# Autodesk Inventor assembly: byk
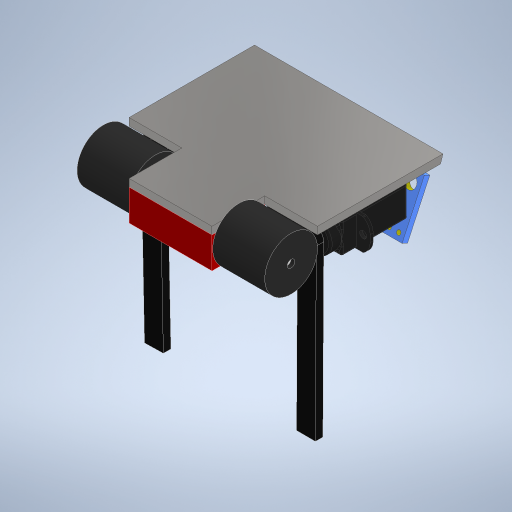
[picture p0: Inventor's stored thumbnail of the model, 512x512]
Saved by Autodesk Inventor 2023 (Build 270158000, 158)
## iProperties
Created: 2023-07-30
Part Number: byk
Document SubType Name: Assembly
Designer: Kamil
Author: Kamil
## Documents named in this file (10)
- C:\Users\Kamil\Documents\Inventor\MikroNalesnik\byk.iam
- C:\Users\Kamil\Documents\Inventor\MikroNalesnik\silnik_2.ipt
- C:\Users\Kamil\Documents\Inventor\MikroNalesnik\spod.ipt
- C:\Users\Kamil\Documents\Inventor\MikroNalesnik\TOF_VL53L0X (1).ipt
- C:\Users\Kamil\Documents\Inventor\MikroNalesnik\servo_mini_1370hd_cos.ipt
- C:\Users\Kamil\Documents\Inventor\MikroNalesnik\kolko.ipt
- C:\Users\Kamil\Documents\Inventor\MikroNalesnik\nozzz.ipt
- C:\Users\Kamil\Documents\Inventor\MikroNalesnik\wach.ipt
- C:\Users\Kamil\Documents\Inventor\MikroNalesnik\uchwyt silnikow.ipt
- C:\Users\Kamil\Documents\Inventor\MikroNalesnik\pcbb.ipt
## Components (15 placed, 9 different names)
1. silnik_2:2 — Zestawiające:21, Zestawiające:23, Zestawiające:25, Zestawiające:26, Zestawiające:27
2. spod:1 — Zestawiające:10, Zestawiające:11, Równoległe:6, Równoległe:7, Równoległe:8, Zestawiające:22, Zestawiające:24, Równoległe:9, Równoległe:12, Kątowe:1, Równoległe:18
3. TOF_VL53L0X (1):1 — Równoległe:3, Zestawiające:8, Równoległe:14, Równoległe:17
4. TOF_VL53L0X (1):2 — Równoległe:3, Równoległe:4, Zestawiające:8, Zestawiające:9, Kątowe:1, Równoległe:14, Równoległe:15, Równoległe:16, Równoległe:17
5. TOF_VL53L0X (1):3 — Równoległe:4, Zestawiające:9, Równoległe:15, Równoległe:16, Równoległe:18
6. servo_mini_1370hd_cos:1 — Zestawiające:10, Równoległe:5, Równoległe:8, Zestawiające:18, Zestawiające:19
7. servo_mini_1370hd_cos:2 — Zestawiające:11, Równoległe:5, Zestawiające:16, Zestawiające:17, Równoległe:7
8. kolko:1
9. nozzz:1 — Równoległe:6
10. wach:1 — Zestawiające:16, Zestawiające:17
11. wach:2 — Zestawiające:18, Zestawiające:19
12. silnik_2:3 — Zestawiające:21, Zestawiające:22, Zestawiające:23
13. kolko:2 — Zestawiające:26, Zestawiające:27
14. uchwyt silnikow:1 — Zestawiające:24, Zestawiające:25, Równoległe:9
15. pcbb:1 — Równoległe:12
## Relationships (29: Mate 15, Flush 13, Angle 1)
- Równoległe:3 [Flush]: TOF_VL53L0X (1):1 ↔ TOF_VL53L0X (1):2
- Równoległe:4 [Flush]: TOF_VL53L0X (1):2 ↔ TOF_VL53L0X (1):3
- Zestawiające:8 [Mate] (5 mm): TOF_VL53L0X (1):1 ↔ TOF_VL53L0X (1):2
- Zestawiające:9 [Mate] (5 mm): TOF_VL53L0X (1):2 ↔ TOF_VL53L0X (1):3
- Zestawiające:10 [Mate]: spod:1 ↔ servo_mini_1370hd_cos:1
- Zestawiające:11 [Mate]: spod:1 ↔ servo_mini_1370hd_cos:2
- Równoległe:5 [Flush]: servo_mini_1370hd_cos:1 ↔ servo_mini_1370hd_cos:2
- Równoległe:6 [Flush]: spod:1 ↔ nozzz:1
- Zestawiające:16 [Mate]: servo_mini_1370hd_cos:2 ↔ wach:1
- Zestawiające:17 [Mate]: servo_mini_1370hd_cos:2 ↔ wach:1
- Równoległe:7 [Flush]: spod:1 ↔ servo_mini_1370hd_cos:2
- Równoległe:8 [Flush]: spod:1 ↔ servo_mini_1370hd_cos:1
- Zestawiające:18 [Mate]: servo_mini_1370hd_cos:1 ↔ wach:2
- Zestawiające:19 [Mate]: servo_mini_1370hd_cos:1 ↔ wach:2
- Zestawiające:21 [Mate] (2 mm): silnik_2:2 ↔ silnik_2:3
- Zestawiające:22 [Mate]: spod:1 ↔ silnik_2:3
- Zestawiające:23 [Mate]: silnik_2:2 ↔ silnik_2:3
- Zestawiające:24 [Mate]: spod:1 ↔ uchwyt silnikow:1
- Zestawiające:25 [Mate]: silnik_2:2 ↔ uchwyt silnikow:1
- Równoległe:9 [Flush]: spod:1 ↔ uchwyt silnikow:1
- Zestawiające:26 [Mate]: silnik_2:2 ↔ kolko:2
- Zestawiające:27 [Mate]: silnik_2:2 ↔ kolko:2
- Równoległe:12 [Flush] (-2 mm): spod:1 ↔ pcbb:1
- Kątowe:1 [Angle] (155 deg): spod:1 ↔ TOF_VL53L0X (1):2
- Równoległe:14 [Flush]: TOF_VL53L0X (1):1 ↔ TOF_VL53L0X (1):2
- Równoległe:15 [Flush]: TOF_VL53L0X (1):2 ↔ TOF_VL53L0X (1):3
- Równoległe:16 [Flush]: TOF_VL53L0X (1):2 ↔ TOF_VL53L0X (1):3
- Równoległe:17 [Flush]: TOF_VL53L0X (1):1 ↔ TOF_VL53L0X (1):2
- Równoległe:18 [Flush]: spod:1 ↔ TOF_VL53L0X (1):3
